# Autodesk Inventor assembly: Disceep20
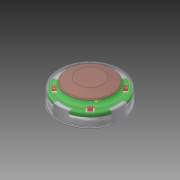
[picture p0: Inventor's stored thumbnail of the model, 180x180]
Saved by Autodesk Inventor 2014 (Build 180170000, 170)
## iProperties
Created: 2014-11-29
Part Number: Disceep20
Document SubType Name: Assembly
Designer: DV
Author: DV
## Documents named in this file (10)
- C:\Users\DV\Documents\github\Disceep\Disceep20.iam
- C:\Users\DV\Documents\github\Disceep\12mmPiezo.ipt
- C:\Users\DV\Documents\github\Disceep\cr1620.ipt
- C:\Users\DV\Documents\github\Allegro_Design_Library\PCB.ipt
- C:\Users\DV\Documents\github\Allegro_Design_Library\NegBattTerminal.ipt
- C:\Users\DV\Documents\github\Disceep\TSSOP_14.iam
- C:\Users\DV\Documents\github\Allegro_Design_Library\PosBatClip.ipt
- C:\Users\DV\Downloads\User Library-LTST-C190EKT (1)\Imported Components\User Library-LTST-C190EKT\Assembly2.iam
- C:\Users\DV\Documents\github\Disceep\Case.ipt
- C:\Users\DV\Documents\github\Disceep\Disceep20CaseBottom.ipt
## Components (15 placed, 9 different names)
1. 12mmPiezo:1 — Mate:6, Insert:1
2. cr1620:1 — Mate:4, Mate:5
3. PCB:1 — Mate:1, Mate:2, Mate:3, Mate:5, Mate:7, Mate:8, Mate:9, Mate:10, Angle:1, Mate:11
4. NegBattTerminal:1 — Mate:1, Mate:2, Mate:3, Mate:4
5. TSSOP_14:1 [sub-assembly] — Mate:7, Angle:2
6. Case:1 — Mate:16, Insert:1, Mate:17
7. Disceep20CaseBottom:1 — Flush:2
8. PosBatClip:1 — Mate:9, Mate:10, Angle:1
9. PosBatClip:2 — Mate:14
10. PosBatClip:3 — Mate:13, Mate:15
11. PosBatClip:4
12. Assembly2:2 [sub-assembly] — Mate:11, Flush:1
13. Assembly2:3 [sub-assembly]
14. Assembly2:4 [sub-assembly] — Mate:17
15. Assembly2:5 [sub-assembly]
## Component patterns: (4 elements, first: PosBatClip:1), (4 elements, first: Assembly2:2)
## Relationships (21: Mate 16, Angle 2, Flush 2, Insert 1)
- Mate:1: PCB:1 ↔ NegBattTerminal:1
- Mate:2: PCB:1 ↔ NegBattTerminal:1
- Mate:3: PCB:1 ↔ NegBattTerminal:1
- Mate:4: cr1620:1 ↔ NegBattTerminal:1
- Mate:5: cr1620:1 ↔ PCB:1
- Mate:6: 12mmPiezo:1
- Mate:7: PCB:1 ↔ TSSOP_14:1
- Mate:8: PCB:1
- Mate:9: PCB:1 ↔ PosBatClip:1
- Mate:10: PCB:1 ↔ PosBatClip:1
- Angle:1 (-15 deg): PCB:1 ↔ PosBatClip:1
- Angle:2 (0 deg): TSSOP_14:1
- Mate:11: PCB:1 ↔ Assembly2:2
- Mate:13: PosBatClip:3
- Mate:14: PosBatClip:2
- Mate:15: PosBatClip:3
- Flush:1 (0.254 mm): Assembly2:2
- Mate:16: Case:1
- Insert:1: 12mmPiezo:1 ↔ Case:1
- Mate:17: Case:1 ↔ Assembly2:4
- Flush:2: Disceep20CaseBottom:1
